# Autodesk Inventor assembly: large_motor_with_gear
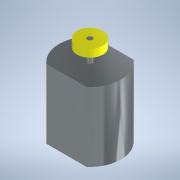
[picture p0: Inventor's stored thumbnail of the model, 180x180]
Saved by Autodesk Inventor 2020 (Build 240168000, 168)
## iProperties
Created: 2021-03-06
Part Number: large_motor_with_gear
Document SubType Name: Assembly
Designer: Harry
Author: Harry
## Documents named in this file (3)
- C:\Users\Harry\Documents\hacktheburgh\octocatch\cad\large_motor_with_gear.iam
- C:\Users\Harry\Documents\hacktheburgh\octocatch\cad\dc_motor_larger.ipt
- C:\Users\Harry\Documents\hacktheburgh\octocatch\cad\belt_gear.ipt
## Components (2 placed, 2 different names)
1. dc_motor_larger:1 — Insert:1
2. belt_gear:1 — Insert:1
## Relationships (1: Insert 1)
- Insert:1: dc_motor_larger:1 ↔ belt_gear:1
